# Autodesk Inventor assembly: noga_pre_MIR1
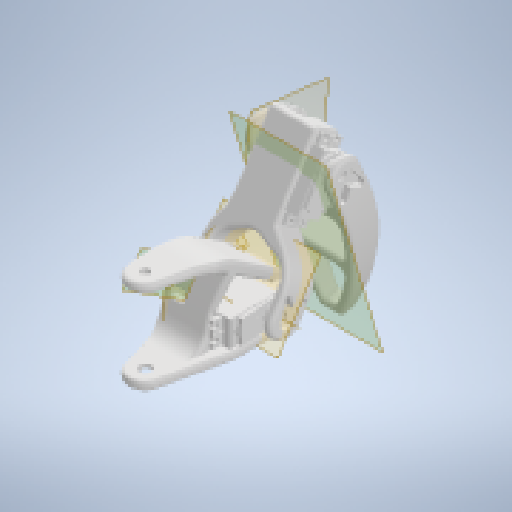
[picture p0: Inventor's stored thumbnail of the model, 512x512]
Saved by Autodesk Inventor 2023.4 (Build 274418000, 418)
## iProperties
Created: 2024-06-27
Part Number: noga_pre_MIR1
Document SubType Name: Assembly
Designer: kamil
Author: kamil
## Documents named in this file (5)
- E:\PROJECTS_REPOS\Robal-2.0\mechanics\noga_pre_MIR1.iam
- E:\PROJECTS_REPOS\Robal-2.0\mechanics\Standard-Servo_MIR3.ipt
- E:\PROJECTS_REPOS\Robal-2.0\mechanics\czlon2_pre_MIR2.ipt
- E:\PROJECTS_REPOS\Robal-2.0\mechanics\czlon3_pre_MIR1.ipt
- E:\PROJECTS_REPOS\Robal-2.0\mechanics\czlon4_pre_2_MIR1.ipt
## Components (5 placed, 4 different names)
1. Standard-Servo_MIR3:1 — Zestawiające:11, Zestawiające:10, Zestawiające:9, Zestawiające:12
2. czlon2_pre_MIR2:1 — Zestawiające:11, Zestawiające:10, Zestawiające:9, Zestawiające:13
3. czlon3_pre_MIR1:1 — Zestawiające:13, Zestawiające:12, Równoległe:4, Zestawiające:21, Zestawiające:17
4. Standard-Servo_MIR3:3 — Równoległe:4, Zestawiające:21, Zestawiające:17, Zestawiające:23, Zestawiające:22
5. czlon4_pre_2_MIR1:1 — Zestawiające:23, Zestawiające:22
## Relationships (10: Mate 9, Flush 1)
- Zestawiające:11 [Mate]: Standard-Servo_MIR3:1 ↔ czlon2_pre_MIR2:1
- Zestawiające:10 [Mate] (1 mm): Standard-Servo_MIR3:1 ↔ czlon2_pre_MIR2:1
- Zestawiające:9 [Mate] (1 mm): Standard-Servo_MIR3:1 ↔ czlon2_pre_MIR2:1
- Zestawiające:13 [Mate]: czlon2_pre_MIR2:1 ↔ czlon3_pre_MIR1:1
- Zestawiające:12 [Mate] (2.1 mm): Standard-Servo_MIR3:1 ↔ czlon3_pre_MIR1:1
- Równoległe:4 [Flush]: czlon3_pre_MIR1:1 ↔ Standard-Servo_MIR3:3
- Zestawiające:21 [Mate]: czlon3_pre_MIR1:1 ↔ Standard-Servo_MIR3:3
- Zestawiające:17 [Mate] (1 mm): czlon3_pre_MIR1:1 ↔ Standard-Servo_MIR3:3
- Zestawiające:23 [Mate]: Standard-Servo_MIR3:3 ↔ czlon4_pre_2_MIR1:1
- Zestawiające:22 [Mate] (2.1 mm): Standard-Servo_MIR3:3 ↔ czlon4_pre_2_MIR1:1
